# Autodesk Inventor assembly: Assembly1
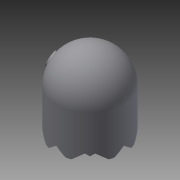
[picture p0: Inventor's stored thumbnail of the model, 180x180]
Saved by Autodesk Inventor 2015 (Build 190159000, 159)
## iProperties
Created: 2015-04-11
Part Number: Assembly1
Document SubType Name: Assembly
Designer: tquinn
Author: tquinn
## Documents named in this file (3)
- Z:\PuckMan\Inventor Models\Assembly1.iam
- Z:\PuckMan\Inventor Models\Ghost1.ipt
- Z:\PuckMan\Inventor Models\GhostEye.ipt
## Components (2 placed, 2 different names)
1. Ghost1:1 — Tangent:1
2. GhostEye:1 — Tangent:1
## Relationships (1: Tangent 1)
- Tangent:1: Ghost1:1 ↔ GhostEye:1
